# Autodesk Inventor assembly: цепь_MIR4_MIR_MIR
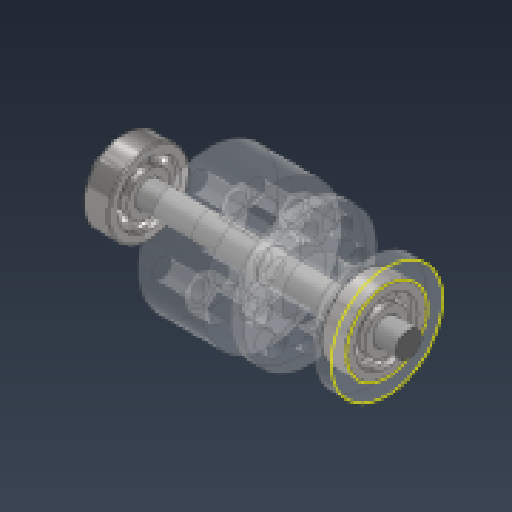
[picture p0: Inventor's stored thumbnail of the model, 512x512]
Saved by Autodesk Inventor 2026 (Build 300175000, 175)
## iProperties
Created: 2024-07-09
Part Number: цепь_MIR4_MIR_MIR
Document SubType Name: Assembly
Designer: Phantom
Author: Phantom
## Documents named in this file (5)
- C:\Users\GameHD\Desktop\Phantom 16950\цепь_MIR4_MIR_MIR.iam
- C:\Users\GameHD\Desktop\Phantom 16950\втулка для подш 2 часть_MIR6_MIR_MIR.ipt
- C:\Users\GameHD\Desktop\Phantom 16950\втулка для подш_MIR6_MIR_MIR.ipt
- C:\Users\GameHD\Desktop\Phantom 16950\Деталь_64_MIR6_MIR_MIR.ipt
- C:\Users\GameHD\Desktop\Phantom 16950\BS 290 SKF - SKF 626-RZ_MIR6_MIR_MIR.ipt
## Components (5 placed, 4 different names)
1. втулка для подш 2 часть_MIR6_MIR_MIR:1 — Совмещение:16, Совмещение:23, Совмещение:20
2. втулка для подш_MIR6_MIR_MIR:1 — Совмещение:16, Совмещение:17
3. Деталь_64_MIR6_MIR_MIR:1 — Совмещение:23, Совмещение:17, Совмещение:21, Совмещение:19
4. BS 290 SKF - SKF 626-RZ_MIR6_MIR_MIR:1 — Совмещение:21, Совмещение:20
5. BS 290 SKF - SKF 626-RZ_MIR6_MIR_MIR:2 — Совмещение:19
## Relationships (6: Mate 6)
- Совмещение:16 [Mate]: втулка для подш 2 часть_MIR6_MIR_MIR:1 ↔ втулка для подш_MIR6_MIR_MIR:1
- Совмещение:23 [Mate]: втулка для подш 2 часть_MIR6_MIR_MIR:1 ↔ Деталь_64_MIR6_MIR_MIR:1
- Совмещение:17 [Mate]: втулка для подш_MIR6_MIR_MIR:1 ↔ Деталь_64_MIR6_MIR_MIR:1
- Совмещение:21 [Mate]: Деталь_64_MIR6_MIR_MIR:1 ↔ BS 290 SKF - SKF 626-RZ_MIR6_MIR_MIR:1
- Совмещение:20 [Mate]: втулка для подш 2 часть_MIR6_MIR_MIR:1 ↔ BS 290 SKF - SKF 626-RZ_MIR6_MIR_MIR:1
- Совмещение:19 [Mate]: Деталь_64_MIR6_MIR_MIR:1 ↔ BS 290 SKF - SKF 626-RZ_MIR6_MIR_MIR:2
